# Autodesk Inventor assembly: x4_Pulley
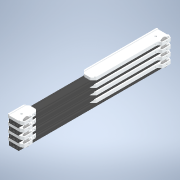
[picture p0: Inventor's stored thumbnail of the model, 180x180]
Saved by Autodesk Inventor 2020 (Build 240168000, 168)
## iProperties
Created: 2020-02-11
Part Number: x4_Pulley
Document SubType Name: Assembly
Designer: maple
Author: maple
## Documents named in this file (2)
- C:\Users\maple\Documents\GitHub\CAD\Robotics 2019-2020\Assembly\PulleySystem\x4_Pulley.iam
- C:\Users\maple\Documents\GitHub\CAD\Robotics 2019-2020\Assembly\PulleySystem\SinglePulley.iam
## Components (4 placed, 1 different names)
1. SinglePulley:1 [sub-assembly] — Mate:1, Flush:1, Flush:2, Flush:3
2. SinglePulley:2 [sub-assembly] — Mate:1, Flush:1, Flush:2, Flush:3, Mate:2, Flush:4, Flush:6, Flush:7
3. SinglePulley:3 [sub-assembly] — Mate:2, Mate:3, Flush:4, Flush:5, Flush:6, Flush:7, Flush:8, Flush:9
4. SinglePulley:4 [sub-assembly] — Mate:3, Flush:5, Flush:8, Flush:9
## Relationships (12: Flush 9, Mate 3)
- Mate:1: SinglePulley:1 ↔ SinglePulley:2
- Flush:1: SinglePulley:1 ↔ SinglePulley:2
- Flush:2: SinglePulley:1 ↔ SinglePulley:2
- Flush:3: SinglePulley:1 ↔ SinglePulley:2
- Mate:2: SinglePulley:2 ↔ SinglePulley:3
- Mate:3: SinglePulley:3 ↔ SinglePulley:4
- Flush:4: SinglePulley:2 ↔ SinglePulley:3
- Flush:5: SinglePulley:3 ↔ SinglePulley:4
- Flush:6: SinglePulley:2 ↔ SinglePulley:3
- Flush:7: SinglePulley:2 ↔ SinglePulley:3
- Flush:8: SinglePulley:3 ↔ SinglePulley:4
- Flush:9: SinglePulley:3 ↔ SinglePulley:4
